# Autodesk Inventor assembly: 可删
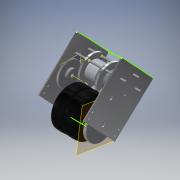
[picture p0: Inventor's stored thumbnail of the model, 180x180]
Saved by Autodesk Inventor 2019 (Build 230136000, 136)
## iProperties
Created: 2020-09-26
Part Number: 可删
Material: 一般
Document SubType Name: Assembly
Designer: zhept
Author: zhept
## Documents named in this file (12)
- C:\Users\zhept\OneDrive\大学\rrst\足回り2020\足回り試作　ゴム車輪\可删.iam
- C:\Users\zhept\OneDrive\大学\rrst\足回り2020\足回り試作　ゴム車輪\KHK_SS0530BOn.ipt
- C:\Users\zhept\OneDrive\大学\rrst\足回り2020\足回り試作　ゴム車輪\モーター RS775-8513DF.iam
- C:\Users\zhept\OneDrive\大学\rrst\足回り2020\足回り試作　ゴム車輪\円 46.9mm.ipt
- C:\Users\zhept\OneDrive\大学\rrst\足回り2020\足回り試作　ゴム車輪\六角スペーサー.ipt
- C:\Users\zhept\OneDrive\大学\rrst\足回り2020\足回り試作　ゴム車輪\円 42.5mm.ipt
- C:\Users\zhept\OneDrive\大学\rrst\足回り2020\足回り試作　ゴム車輪\板.ipt
- C:\Users\zhept\OneDrive\大学\rrst\足回り2020\足回り試作　ゴム車輪\円柱5mm.ipt
- C:\Users\zhept\OneDrive\大学\rrst\足回り2020\HAMMER_CASTER_425ER100\HAMMER_CASTER_425ER100.ipt
- C:\Users\zhept\OneDrive\大学\rrst\足回り2020\KHK_SS05120AOn\KHK_SS05120AOn.ipt
- C:\Users\zhept\OneDrive\大学\rrst\足回り2020\KHK_SSG0840BOn\KHK_SSG0840BOn.ipt
- C:\Users\zhept\OneDrive\大学\rrst\足回り2020\KHK_SS08100AOn\KHK_SS08100AOn.ipt
## Components (16 placed, 11 different names)
1. KHK_SS0530BOn:1 — フラッシュ:2, メイト:1, 回転:1, フラッシュ:3
2. モーター RS775-8513DF:1 [sub-assembly] — 回転:1, メイト:9, 回転:2, 回転:3, メイト:10
3. 円 46.9mm:1 — メイト:9, 挿入:5, メイト:12
4. 六角スペーサー:1 — 回転:3, 挿入:2
5. 六角スペーサー:2 — 回転:2, 挿入:3
6. 円 42.5mm:1 — メイト:10, 挿入:5
7. 板:1 — 挿入:2, 挿入:3, 挿入:4, 角度:1, メイト:12, 挿入:6, 挿入:7, 挿入:8, メイト:14, メイト:18
8. 板:2 — 挿入:4, 角度:1, メイト:22, メイト:24
9. 円柱5mm:1 — 挿入:6
10. 円柱5mm:2 — 挿入:8
11. 円柱5mm:3 — 挿入:7
12. HAMMER_CASTER_425ER100:1 — メイト:13, 角度:2
13. HAMMER_CASTER_425ER100:2 — メイト:13, 角度:2, メイト:15
14. KHK_SS05120AOn:1 — メイト:17, フラッシュ:3
15. KHK_SSG0840BOn:1 — メイト:20, メイト:22
16. KHK_SS08100AOn:1 — メイト:23, メイト:24
## Relationships (31: Mate 17, Insert 7, RevoluteJoint 3, Flush 2, Angle 2)
- フラッシュ:2 [Flush]: KHK_SS0530BOn:1
- メイト:1 [Mate]: KHK_SS0530BOn:1
- 回転:1 [RevoluteJoint]: KHK_SS0530BOn:1 ↔ モーター RS775-8513DF:1
- メイト:9 [Mate]: モーター RS775-8513DF:1 ↔ 円 46.9mm:1
- 回転:2 [RevoluteJoint]: モーター RS775-8513DF:1 ↔ 六角スペーサー:2
- 回転:3 [RevoluteJoint]: モーター RS775-8513DF:1 ↔ 六角スペーサー:1
- メイト:10 [Mate]: モーター RS775-8513DF:1 ↔ 円 42.5mm:1
- 挿入:2 [Insert]: 六角スペーサー:1 ↔ 板:1
- 挿入:3 [Insert]: 六角スペーサー:2 ↔ 板:1
- 挿入:4 [Insert] (115 mm): 板:1 ↔ 板:2
- 角度:1 [Angle] (0 deg): 板:1 ↔ 板:2
- 挿入:5 [Insert] (45 mm): 円 46.9mm:1 ↔ 円 42.5mm:1
- メイト:12 [Mate] (28.5 mm): 円 46.9mm:1 ↔ 板:1
- 挿入:6 [Insert] (-5 mm): 板:1 ↔ 円柱5mm:1
- 挿入:7 [Insert] (-5 mm): 板:1 ↔ 円柱5mm:3
- 挿入:8 [Insert] (-5 mm): 板:1 ↔ 円柱5mm:2
- メイト:13 [Mate]: HAMMER_CASTER_425ER100:1 ↔ HAMMER_CASTER_425ER100:2
- 角度:2 [Angle] (0 deg): HAMMER_CASTER_425ER100:1 ↔ HAMMER_CASTER_425ER100:2
- メイト:14 [Mate]: 板:1
- メイト:15 [Mate]: HAMMER_CASTER_425ER100:2
- メイト:16 [Mate]
- メイト:17 [Mate]: KHK_SS05120AOn:1
- メイト:18 [Mate]: 板:1
- メイト:19 [Mate]
- フラッシュ:3 [Flush]: KHK_SS0530BOn:1 ↔ KHK_SS05120AOn:1
- メイト:20 [Mate]: KHK_SSG0840BOn:1
- メイト:21 [Mate]
- メイト:22 [Mate] (2 mm): 板:2 ↔ KHK_SSG0840BOn:1
- メイト:23 [Mate]: KHK_SS08100AOn:1
- メイト:24 [Mate] (2 mm): 板:2 ↔ KHK_SS08100AOn:1
- メイト:25 [Mate]
